# Autodesk Inventor assembly: DisplayDummyAuschnitt
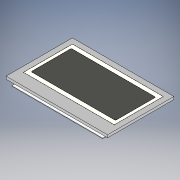
[picture p0: Inventor's stored thumbnail of the model, 180x180]
Saved by Autodesk Inventor 2017 (Build 210142000, 142)
## iProperties
Part Number: DisplayDummyAuschnitt
Material: Generisch
Document SubType Name: Assembly
Designer: aXe
Author: aXe
## Documents named in this file (5)
- C:\Users\aXe\Dropbox\Elektronik\aXe_Dashboard240XL\Gehäuse\DisplayDummyAuschnitt.iam
- C:\Users\aXe\Dropbox\Elektronik\aXe_Dashboard240XL\Gehäuse\DisplayDummy.ipt
- C:\Users\aXe\Dropbox\Elektronik\aXe_Dashboard240XL\Gehäuse\DummyAuschnitt.ipt
- C:\Users\aXe\Dropbox\Elektronik\aXe_Dashboard240XL\Gehäuse\Auschnitt2.ipt
- F:\DummyAuschnitt2.ipt
## Components (4 placed, 4 different names)
1. DisplayDummy:1 — Fluchtend:1, Fluchtend:2, Fluchtend:3, Fluchtend:4, Fluchtend:5, Fluchtend:6, Passend:1, Passend:2
2. DummyAuschnitt:1 — Fluchtend:1, Fluchtend:2, Fluchtend:3
3. Auschnitt2:1 — Fluchtend:4, Fluchtend:5
4. DummyAuschnitt2:1 — Fluchtend:6, Passend:1, Passend:2
## Relationships (8: Flush 6, Mate 2)
- Fluchtend:1 [Flush]: DisplayDummy:1 ↔ DummyAuschnitt:1
- Fluchtend:2 [Flush]: DisplayDummy:1 ↔ DummyAuschnitt:1
- Fluchtend:3 [Flush]: DisplayDummy:1 ↔ DummyAuschnitt:1
- Fluchtend:4 [Flush]: DisplayDummy:1 ↔ Auschnitt2:1
- Fluchtend:5 [Flush]: DisplayDummy:1 ↔ Auschnitt2:1
- Fluchtend:6 [Flush]: DisplayDummy:1 ↔ DummyAuschnitt2:1
- Passend:1 [Mate] (0.1 mm): DisplayDummy:1 ↔ DummyAuschnitt2:1
- Passend:2 [Mate] (0.1 mm): DisplayDummy:1 ↔ DummyAuschnitt2:1
